# Autodesk Inventor assembly: Minifix D15
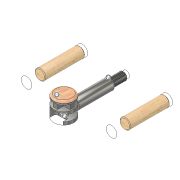
[picture p0: Inventor's stored thumbnail of the model, 180x180]
Saved by Autodesk Inventor 2022 (Build 260153000, 153)
## iProperties
RuleStatus: InUse
Created: 2021-04-12
Part Number: Minifix D15
Document SubType Name: Assembly
Designer: SauliusD
Author: SauliusD
## iProperties of the stored document MemberDocs/xBhionitrLskg5okcLmbhxzpq0d
RuleStatus: InUse
Created: 2021-04-12
Part Number: Minifix D15
Document SubType Name: Assembly
Designer: SauliusD
Author: SauliusD
## iProperties of the stored document MemberDocs/x21vfl24nEsbwj5utJmmzwgz5Zg
RuleStatus: InUse
Created: 2021-04-12
Part Number: Minifix D15
Document SubType Name: Assembly
Designer: SauliusD
Author: SauliusD
## iProperties of the stored document MemberDocs/x0jdcevhzLcwmmdi3Galxdgoq2f
RuleStatus: InUse
Created: 2021-04-12
Part Number: Minifix D15
Document SubType Name: Assembly
Designer: SauliusD
Author: SauliusD
## iProperties of the stored document MemberDocs/x5bjl4dsfGse4k2cmR5mpcu4fTb
RuleStatus: InUse
Created: 2021-04-12
Part Number: Minifix D15
Document SubType Name: Assembly
Designer: SauliusD
Author: SauliusD
## iProperties of the stored document MemberDocs/xIjj22hbeEceu35k0JrjrwbsbPf
RuleStatus: InUse
Created: 2021-04-12
Part Number: Minifix D15
Document SubType Name: Assembly
Designer: SauliusD
Author: SauliusD
## iProperties of the stored document MemberDocs/xF21nqvzwOssqtdd0XdgrfqbxVc
RuleStatus: InUse
Created: 2021-04-12
Part Number: Minifix D15
Document SubType Name: Assembly
Designer: SauliusD
Author: SauliusD
## iProperties of the stored document MemberDocs/xBhsho1pzI0sfvepy3clxzwog5c
RuleStatus: InUse
Created: 2021-04-12
Part Number: Minifix D15
Document SubType Name: Assembly
Designer: SauliusD
Author: SauliusD
## iProperties of the stored document MemberDocs/xGxftdgamIcpm5xvwEtm5u4h4Mg
RuleStatus: InUse
Created: 2021-04-12
Part Number: Minifix D15
Document SubType Name: Assembly
Designer: SauliusD
Author: SauliusD
## iProperties of the stored document MemberDocs/xNvpyk0tfN0vnhcu5LnihwwonHb
RuleStatus: InUse
Created: 2021-04-12
Part Number: Minifix D15
Document SubType Name: Assembly
Designer: SauliusD
Author: SauliusD
## iProperties of the stored document MemberDocs/xMrtnr0ojO01dqi1sRxgterhoWh
RuleStatus: InUse
Created: 2021-04-12
Part Number: Minifix D15
Document SubType Name: Assembly
Designer: SauliusD
Author: SauliusD
## iProperties of the stored document MemberDocs/xKss25ezeEcbqc25nYflf1cs2Sd
RuleStatus: InUse
Created: 2021-04-12
Part Number: Minifix D15
Document SubType Name: Assembly
Designer: SauliusD
Author: SauliusD
## iProperties of the stored document MemberDocs/xNpg0sqpdDswitbpk4ulpjf1r4g
RuleStatus: InUse
Created: 2021-04-12
Part Number: Minifix D15
Document SubType Name: Assembly
Designer: SauliusD
Author: SauliusD
## iProperties of the stored document MemberDocs/xS02vi10fPkd5szyhJrdlwct0Nd
RuleStatus: InUse
Created: 2021-04-12
Part Number: Minifix D15
Document SubType Name: Assembly
Designer: SauliusD
Author: SauliusD
## iProperties of the stored document MemberDocs/xPmqb5ddxF0uq0u5oLhe5m4eeKd
RuleStatus: InUse
Created: 2021-04-12
Part Number: Minifix D15
Document SubType Name: Assembly
Designer: SauliusD
Author: SauliusD
## iProperties of the stored document MemberDocs/xWpht4v4dBkll3xkv35o5zhuiZb
RuleStatus: InUse
Created: 2021-04-12
Part Number: Minifix D15
Document SubType Name: Assembly
Designer: SauliusD
Author: SauliusD
## iProperties of the stored document MemberDocs/xZ1c2ba2mM0lmxkrvSro5da255c
RuleStatus: InUse
Created: 2021-04-12
Part Number: Minifix D15
Document SubType Name: Assembly
Designer: SauliusD
Author: SauliusD
## Documents named in this file (17)
- C:\W4INV 2024 Design\PROJECTS\MODEL STATE LIBRARY COMPONENTS\Minifix D15\Minifix D15.iam
- C:\W4INV 2021 Design\PROJECTS\Inventor 2022\Minifix D15\Parts\Minifix D15 V4.ipt
- C:\W4INV 2021 Design\PROJECTS\Inventor 2022\Minifix D15\Parts\Connecting Pin.ipt
- C:\W4INV 2021 Design\PROJECTS\Inventor 2022\Minifix D15\Parts\Dowel.ipt
- C:\W4INV 2021 Design\PROJECTS\Inventor 2022\Minifix D15\Parts\Minifix Cap.ipt
- C:\W4INV 2024 Design\PROJECTS\MODEL STATE LIBRARY COMPONENTS\Minifix D15\Parts\Minifix D15 V4.ipt
- C:\W4INV 2024 Design\PROJECTS\MODEL STATE LIBRARY COMPONENTS\Minifix D15\Parts\Connecting Pin.ipt
- C:\W4INV 2024 Design\PROJECTS\MODEL STATE LIBRARY COMPONENTS\Minifix D15\Parts\Dowel.ipt
- C:\W4INV 2024 Design\PROJECTS\MODEL STATE LIBRARY COMPONENTS\Minifix D15\Parts\Minifix Cap.ipt
- C:\W4INV 2022 Design\LIBRARY\Fixed joints\Minifix joint\Minifix D15\Parts\Minifix D15 V4.ipt
- C:\W4INV 2022 Design\LIBRARY\Fixed joints\Minifix joint\Minifix D15\Parts\Connecting Pin.ipt
- C:\W4INV 2022 Design\LIBRARY\Fixed joints\Minifix joint\Minifix D15\Parts\Dowel.ipt
- C:\W4INV 2022 Design\LIBRARY\Fixed joints\Minifix joint\Minifix D15\Parts\Minifix Cap.ipt
- C:\W4INV 2022 Design\PROJECTS\MODEL STATE LIBRARY COMPONENTS\Minifix D15\Parts\Minifix D15 V4.ipt
- C:\W4INV 2022 Design\PROJECTS\MODEL STATE LIBRARY COMPONENTS\Minifix D15\Parts\Connecting Pin.ipt
- C:\W4INV 2022 Design\PROJECTS\MODEL STATE LIBRARY COMPONENTS\Minifix D15\Parts\Dowel.ipt
- C:\W4INV 2022 Design\PROJECTS\MODEL STATE LIBRARY COMPONENTS\Minifix D15\Parts\Minifix Cap.ipt
## Components (5 placed, 4 different names)
1. Minifix D15 V4:1 — Mate:1, Insert:1
2. Connecting Pin:1 — Mate:2, Mate:1, Mate:3, Mate:4, Mate:6, Mate:7, Flush:1
3. Dowel:1 — Mate:3, Mate:4, Mate:5
4. Dowel:2 — Mate:6, Mate:7, Flush:1
5. Minifix Cap:1 — Insert:1
## Relationships (9: Mate 7, Flush 1, Insert 1)
- Mate:2: Connecting Pin:1
- Mate:1: Minifix D15 V4:1 ↔ Connecting Pin:1
- Mate:3: Connecting Pin:1 ↔ Dowel:1
- Mate:4: Connecting Pin:1 ↔ Dowel:1
- Mate:5 (32 mm): Dowel:1
- Mate:6: Connecting Pin:1 ↔ Dowel:2
- Mate:7: Connecting Pin:1 ↔ Dowel:2
- Flush:1 (-32 mm): Connecting Pin:1 ↔ Dowel:2
- Insert:1: Minifix D15 V4:1 ↔ Minifix Cap:1
## Named parameters: Connecting_Pin_Length = 34 mm, iTrigger0 = 0
